# Autodesk Inventor assembly: Turret Assembly
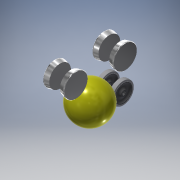
[picture p0: Inventor's stored thumbnail of the model, 180x180]
Saved by Autodesk Inventor 2019.4 (Build 234330000, 330)
## iProperties
Created: 2020-01-16
Part Number: Turret Assembly
Document SubType Name: Assembly
Designer: admin
Author: admin
## Documents named in this file (4)
- C:\Users\admin\Desktop\FRC 2020 Engineering\GitHub\7738-2020\Robot V2\Turret\Turret Assembly.iam
- C:\Users\admin\Desktop\FRC 2020 Engineering\GitHub\7738-2020\Robot V2\Turret\Flywheel Half.ipt
- C:\Users\admin\Desktop\FRC 2020 Engineering\GitHub\7738-2020\Power Cell.ipt
- C:\Users\admin\Desktop\FRC 2020 Engineering\GitHub\7738-2020\Robot V2\Turret\Colson_Performa_4_x_0_875_1_2_Hex_bore_217-4049.ipt
## Components (7 placed, 3 different names)
1. Power Cell:1 — Mate:3
2. Flywheel Half:3 — Mate:11
3. Flywheel Half:4 — Mate:9, Mate:10
4. Colson_Performa_4_x_0_875_1_2_Hex_bore_217-4049:1 — Mate:12, Mate:14, Mate:15, Mate:16
5. Colson_Performa_4_x_0_875_1_2_Hex_bore_217-4049:2 — Mate:15, Mate:16, Mate:17
6. Flywheel Half:5 — Mate:20, Mate:21, Mate:22
7. Flywheel Half:6
## Relationships (16: Mate 16)
- Mate:3: Power Cell:1
- [Mate] (50 mm): Flywheel Half:3 ↔ Flywheel Half:4
- [Mate]: Flywheel Half:3 ↔ Flywheel Half:4
- Mate:9 (25 mm): Flywheel Half:4
- Mate:10 (-114.3 mm): Flywheel Half:4
- Mate:11 (150 mm): Flywheel Half:3
- Mate:12 (114.3 mm): Colson_Performa_4_x_0_875_1_2_Hex_bore_217-4049:1
- Mate:14: Colson_Performa_4_x_0_875_1_2_Hex_bore_217-4049:1
- Mate:15 (40 mm): Colson_Performa_4_x_0_875_1_2_Hex_bore_217-4049:1 ↔ Colson_Performa_4_x_0_875_1_2_Hex_bore_217-4049:2
- Mate:16: Colson_Performa_4_x_0_875_1_2_Hex_bore_217-4049:1 ↔ Colson_Performa_4_x_0_875_1_2_Hex_bore_217-4049:2
- Mate:17 (20 mm): Colson_Performa_4_x_0_875_1_2_Hex_bore_217-4049:2
- [Mate] (50 mm): Flywheel Half:5 ↔ Flywheel Half:6
- [Mate]: Flywheel Half:5 ↔ Flywheel Half:6
- Mate:20 (116.84 mm): Flywheel Half:5
- Mate:21 (25 mm): Flywheel Half:5
- Mate:22 (150 mm): Flywheel Half:5
## Named parameters: d8_d0 = 50 mm, d9_d1 = 0 mm, d19_d8_d0 = 50 mm, d20_d9_d1 = 0 mm
